# Autodesk Inventor assembly: P1704_E2
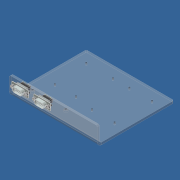
[picture p0: Inventor's stored thumbnail of the model, 180x180]
Saved by Autodesk Inventor 2015 SP2 (Build 190223200, 223)
## iProperties
Created: 2018-05-15
Part Number: P1704_E2
Project: Manette arcade
Description: Console
Document SubType Name: Assembly
Designer: Alexandre.PICOTTE
Author: Alexandre.PICOTTE
## Documents named in this file (4)
- C:\Users\Alexandre.PICOTTE\Documents\P1704_Manettes\06_Dessins\Manette_arcade\P1704_E2_Console.iam
- C:\Users\Alexandre.PICOTTE\Documents\P1704_Manettes\06_Dessins\Manette_arcade\P1704_007_Plaque.ipt
- C:\Users\Alexandre.PICOTTE\Documents\Inventor\Content Center Files\R2015\fr-FR\D-Sub Male Crimp\D-Sub Male Crimp 9CKT.ipt
- C:\Users\Alexandre.PICOTTE\Documents\Inventor\Content Center Files\R2015\fr-FR\ISO 4762(2)\ISO 4762 - M3 x 5ISO.ipt
## Components (7 placed, 3 different names)
1. P1704_007_Plaque:1 — Placage:1, Placage:2, Placage:3, Placage:4, Angle:1, Angle:2
2. Sertissage mâle D-Sub D-Sub Male Crimp 9CKT:1 — Placage:1, Placage:3, Angle:1, Logement:1, Logement:2
3. Sertissage mâle D-Sub D-Sub Male Crimp 9CKT:2 — Placage:2, Placage:4, Angle:2, Logement:3, Logement:4
4. ISO 4762 M3 x 5:1 — Logement:1
5. ISO 4762 M3 x 5:2 — Logement:2
6. ISO 4762 M3 x 5:3 — Logement:3
7. ISO 4762 M3 x 5:4 — Logement:4
## Relationships (10: Mate 4, Insert 4, Angle 2)
- Placage:1 [Mate]: P1704_007_Plaque:1 ↔ Sertissage mâle D-Sub D-Sub Male Crimp 9CKT:1
- Placage:2 [Mate]: P1704_007_Plaque:1 ↔ Sertissage mâle D-Sub D-Sub Male Crimp 9CKT:2
- Placage:3 [Mate]: P1704_007_Plaque:1 ↔ Sertissage mâle D-Sub D-Sub Male Crimp 9CKT:1
- Placage:4 [Mate]: P1704_007_Plaque:1 ↔ Sertissage mâle D-Sub D-Sub Male Crimp 9CKT:2
- Angle:1 (0 deg): P1704_007_Plaque:1 ↔ Sertissage mâle D-Sub D-Sub Male Crimp 9CKT:1
- Angle:2 (0 deg): P1704_007_Plaque:1 ↔ Sertissage mâle D-Sub D-Sub Male Crimp 9CKT:2
- Logement:1 [Insert]: Sertissage mâle D-Sub D-Sub Male Crimp 9CKT:1 ↔ ISO 4762 M3 x 5:1
- Logement:2 [Insert]: Sertissage mâle D-Sub D-Sub Male Crimp 9CKT:1 ↔ ISO 4762 M3 x 5:2
- Logement:3 [Insert]: Sertissage mâle D-Sub D-Sub Male Crimp 9CKT:2 ↔ ISO 4762 M3 x 5:3
- Logement:4 [Insert]: Sertissage mâle D-Sub D-Sub Male Crimp 9CKT:2 ↔ ISO 4762 M3 x 5:4
